# Autodesk Inventor assembly: CandleHolder-0
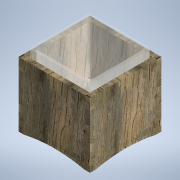
[picture p0: Inventor's stored thumbnail of the model, 180x180]
Saved by Autodesk Inventor 2021 (Build 250183000, 183)
## iProperties
Created: 2016-10-20
Part Number: CandleHolder-0
Document SubType Name: Assembly
Designer: andrew
Author: andrew
## Documents named in this file (4)
- D:\OneDrive\3D Models\CandleHolder\CandleHolder-0.iam
- D:\OneDrive\3D Models\CandleHolder\CandleHolder-1.ipt
- D:\OneDrive\3D Models\CandleHolder\CandleHolder-2.ipt
- D:\OneDrive\3D Models\CandleHolder\CandleHolder-3.ipt
## Components (6 placed, 3 different names)
1. CandleHolder-1:1 — Mate:1, Mate:2, Flush:1, Mate:3, Flush:2, Flush:3, Mate:6
2. CandleHolder-3:1 — Mate:4, Mate:5, Mate:6
3. CandleHolder-2:4 — Mate:3, Flush:2, Flush:3
4. CandleHolder-2:5
5. CandleHolder-2:6
6. CandleHolder-2:7
## Component patterns: (4 elements, first: CandleHolder-2:4)
## Relationships (9: Mate 6, Flush 3)
- Mate:1: CandleHolder-1:1
- Mate:2: CandleHolder-1:1
- Flush:1: CandleHolder-1:1
- Mate:3: CandleHolder-1:1 ↔ CandleHolder-2:4
- Flush:2 (6.35 mm): CandleHolder-1:1 ↔ CandleHolder-2:4
- Flush:3: CandleHolder-1:1 ↔ CandleHolder-2:4
- Mate:4: CandleHolder-3:1
- Mate:5: CandleHolder-3:1
- Mate:6: CandleHolder-1:1 ↔ CandleHolder-3:1
